# Autodesk Inventor assembly: ensamble caja
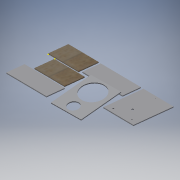
[picture p0: Inventor's stored thumbnail of the model, 180x180]
Saved by Autodesk Inventor 2018 (Build 220112000, 112)
## iProperties
Created: 2019-02-27
Part Number: ensamble caja
Material: Genérico
Document SubType Name: Assembly
Designer: USUARIO WINDOWS
Author: USUARIO WINDOWS
## Documents named in this file (5)
- D:\Projects\Amplificador 1W\ensamble caja.iam
- D:\Projects\Amplificador 1W\frontal.ipt
- D:\Projects\Amplificador 1W\inferior y superior.ipt
- D:\Projects\Amplificador 1W\laterales.ipt
- D:\Projects\Amplificador 1W\trasera.ipt
## Components (6 placed, 4 different names)
1. frontal:1 — Nivelación:2
2. inferior y superior:1 — Nivelación:1, Nivelación:2, Nivelación:3, Nivelación:4, Nivelación:5
3. laterales:1 — Nivelación:5
4. laterales:2 — Nivelación:1
5. inferior y superior:2 — Nivelación:3
6. trasera:1 — Nivelación:4
## Relationships (5: Flush 5)
- Nivelación:1 [Flush]: inferior y superior:1 ↔ laterales:2
- Nivelación:2 [Flush]: frontal:1 ↔ inferior y superior:1
- Nivelación:3 [Flush]: inferior y superior:1 ↔ inferior y superior:2
- Nivelación:4 [Flush]: inferior y superior:1 ↔ trasera:1
- Nivelación:5 [Flush]: inferior y superior:1 ↔ laterales:1
